# Autodesk Inventor assembly: SupportPourCables
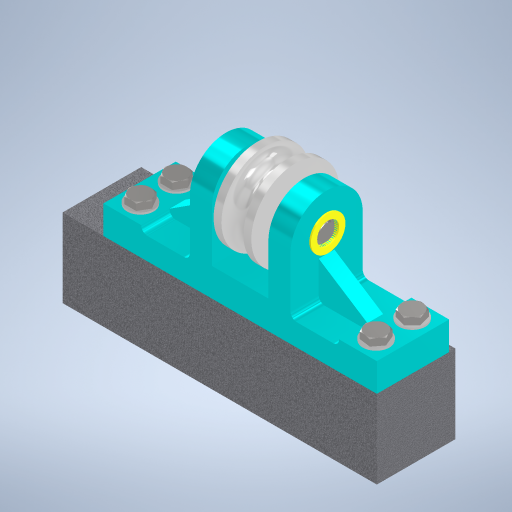
[picture p0: Inventor's stored thumbnail of the model, 512x512]
Saved by Autodesk Inventor 2023.2 (Build 272271030, 271C)
## iProperties
Created: 2023-03-24
Part Number: SupportPourCables
Document SubType Name: Assembly
Designer: Luis Valente
Author: Luis Valente
## Documents named in this file (8)
- C:\Users\lc010\OneDrive\Documentos\Henallux\Inventor School\Support pour Cables\SupportPourCables.iam
- C:\Users\lc010\OneDrive\Documentos\Henallux\Inventor School\Support pour Cables\Socle.ipt
- C:\Users\lc010\OneDrive\Documentos\Henallux\Inventor School\Support pour Cables\Semelle.ipt
- C:\Users\lc010\OneDrive\Documentos\Henallux\Inventor School\Support pour Cables\Roue.ipt
- C:\Users\lc010\OneDrive\Documentos\Henallux\Inventor School\Support pour Cables\Stub.ipt
- C:\Users\lc010\OneDrive\Documentos\Henallux\Inventor School\Support pour Cables\Coussinets.ipt
- C:\Users\lc010\OneDrive\Documentos\Inventor\Content Center Files\R2023\en-US\AS 1237 (3.1)\AS 1237 - 8 mm(1)Aluminium-6061.ipt
- C:\Users\lc010\OneDrive\Documentos\Inventor\Content Center Files\R2023\en-US\AS 1111\AS 1111 - M8 x 40.ipt
## Components (14 placed, 7 different names)
1. Socle:1 — Mate:1, Mate:2
2. Semelle:1 — Mate:1, Mate:2, Rotational:1, Rotational:2, Insert:5, Insert:6, Insert:7, Insert:8, Insert:9, Insert:10, Mate:3, Mate:4, Mate:5, Mate:6, Mate:7, Mate:8, Mate:9, Mate:10
3. Roue:1 — Rotational:1, Rotation:1
4. Stub:1 — Rotational:2, Rotation:1
5. Coussinets:1 — Insert:5
6. Coussinets:2 — Insert:6
7. AS 1237 (3.1) 8 mm - Aluminum 6061:1 — Mate:3, Mate:4, Rotation:2
8. AS 1237 (3.1) 8 mm - Aluminum 6061:2 — Mate:5, Mate:6
9. AS 1237 (3.1) 8 mm - Aluminum 6061:3 — Mate:7, Mate:8
10. AS 1237 (3.1) 8 mm - Aluminum 6061:4 — Mate:9, Mate:10
11. AS 1111 - Metric M8 x 40:1 — Insert:7, Rotation:2
12. AS 1111 - Metric M8 x 40:3 — Insert:8
13. AS 1111 - Metric M8 x 40:2 — Insert:9
14. AS 1111 - Metric M8 x 40:4 — Insert:10
## Relationships (20: Mate 10, Insert 6, RevoluteJoint 2, RelateRotation 2)
- Mate:1: Socle:1 ↔ Semelle:1
- Mate:2: Socle:1 ↔ Semelle:1
- Rotational:1 [RevoluteJoint] (2 mm): Semelle:1 ↔ Roue:1
- Rotational:2 [RevoluteJoint]: Semelle:1 ↔ Stub:1
- Rotation:1 [RelateRotation] (1.857 ul): Roue:1 ↔ Stub:1
- Insert:5: Semelle:1 ↔ Coussinets:1
- Insert:6: Semelle:1 ↔ Coussinets:2
- Insert:7: Semelle:1 ↔ AS 1111 - Metric M8 x 40:1
- Insert:8: Semelle:1 ↔ AS 1111 - Metric M8 x 40:3
- Insert:9: Semelle:1 ↔ AS 1111 - Metric M8 x 40:2
- Insert:10: Semelle:1 ↔ AS 1111 - Metric M8 x 40:4
- Mate:3: Semelle:1 ↔ AS 1237 (3.1) 8 mm - Aluminum 6061:1
- Mate:4: Semelle:1 ↔ AS 1237 (3.1) 8 mm - Aluminum 6061:1
- Mate:5: Semelle:1 ↔ AS 1237 (3.1) 8 mm - Aluminum 6061:2
- Mate:6: Semelle:1 ↔ AS 1237 (3.1) 8 mm - Aluminum 6061:2
- Mate:7: Semelle:1 ↔ AS 1237 (3.1) 8 mm - Aluminum 6061:3
- Mate:8: Semelle:1 ↔ AS 1237 (3.1) 8 mm - Aluminum 6061:3
- Mate:9: Semelle:1 ↔ AS 1237 (3.1) 8 mm - Aluminum 6061:4
- Mate:10: Semelle:1 ↔ AS 1237 (3.1) 8 mm - Aluminum 6061:4
- Rotation:2 [RelateRotation] (1 ul): AS 1237 (3.1) 8 mm - Aluminum 6061:1 ↔ AS 1111 - Metric M8 x 40:1
